# Autodesk Inventor assembly: test
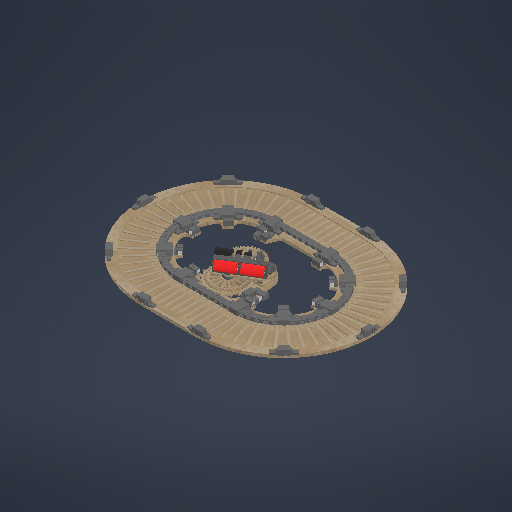
[picture p0: Inventor's stored thumbnail of the model, 512x512]
Saved by Autodesk Inventor 2026.1 (Build 301233020, 233B)
## iProperties
Created: 2025-09-27
Part Number: test
Document SubType Name: Assembly
Designer: hibik
Author: hibik
## Documents named in this file (4)
- C:\Users\hibik\Documents\Robomech\conveyer\All_body.iam
- C:\Users\hibik\Documents\Robomech\conveyer\power_module\Assy_power_module.iam
- C:\Users\hibik\Documents\Robomech\conveyer\liniar_module\linear_module_test.iam
- C:\Users\hibik\Documents\Robomech\conveyer\curve_module\curve_module_test.iam
## Components (11 placed, 3 different names)
1. Assy_power_module:1 [sub-assembly] — フラッシュ:1, 挿入:1, フラッシュ:2, フラッシュ:3
2. linear_module_test:1 [sub-assembly] — 挿入:1, 角度:1, メイト:17, メイト:18, フラッシュ:12
3. curve_module_test:1 [sub-assembly] — メイト:5, メイト:6, フラッシュ:6, メイト:17, メイト:18, フラッシュ:12
4. curve_module_test:2 [sub-assembly] — メイト:5, メイト:6, フラッシュ:6, メイト:9, メイト:10, フラッシュ:8
5. curve_module_test:3 [sub-assembly] — メイト:9, メイト:10, フラッシュ:8
6. curve_module_test:4 [sub-assembly] — メイト:21, メイト:22, フラッシュ:14
7. curve_module_test:5 [sub-assembly] — メイト:19, メイト:20, フラッシュ:13
8. curve_module_test:6 [sub-assembly]
9. curve_module_test:7 [sub-assembly]
10. curve_module_test:8 [sub-assembly]
11. linear_module_test:4 [sub-assembly] — メイト:19, メイト:20, フラッシュ:13, メイト:21, メイト:22, フラッシュ:14
## Relationships (32: Mate 18, Flush 12, Insert 1, Angle 1)
- フラッシュ:1 [Flush]: Assy_power_module:1
- 挿入:1 [Insert] (2.5 mm): Assy_power_module:1 ↔ linear_module_test:1
- 角度:1 [Angle] (0 deg): linear_module_test:1
- フラッシュ:2 [Flush]: Assy_power_module:1
- フラッシュ:3 [Flush]: Assy_power_module:1
- メイト:5 [Mate] (0.5 mm): curve_module_test:1 ↔ curve_module_test:2
- メイト:6 [Mate] (0.5 mm): curve_module_test:1 ↔ curve_module_test:2
- フラッシュ:6 [Flush]: curve_module_test:1 ↔ curve_module_test:2
- [Mate] (0.5 mm): curve_module_test:3 ↔ curve_module_test:4
- [Mate] (0.5 mm): curve_module_test:3 ↔ curve_module_test:4
- [Flush]: curve_module_test:3 ↔ curve_module_test:4
- メイト:9 [Mate] (0.5 mm): curve_module_test:2 ↔ curve_module_test:3
- メイト:10 [Mate] (0.5 mm): curve_module_test:2 ↔ curve_module_test:3
- フラッシュ:8 [Flush]: curve_module_test:2 ↔ curve_module_test:3
- [Mate] (0.5 mm): curve_module_test:5 ↔ curve_module_test:6
- [Mate] (0.5 mm): curve_module_test:5 ↔ curve_module_test:6
- [Flush]: curve_module_test:5 ↔ curve_module_test:6
- [Mate] (0.5 mm): curve_module_test:7 ↔ curve_module_test:8
- [Mate] (0.5 mm): curve_module_test:7 ↔ curve_module_test:8
- [Flush]: curve_module_test:7 ↔ curve_module_test:8
- [Mate] (0.5 mm): curve_module_test:6 ↔ curve_module_test:7
- [Mate] (0.5 mm): curve_module_test:6 ↔ curve_module_test:7
- [Flush]: curve_module_test:6 ↔ curve_module_test:7
- メイト:17 [Mate]: linear_module_test:1 ↔ curve_module_test:1
- メイト:18 [Mate]: linear_module_test:1 ↔ curve_module_test:1
- フラッシュ:12 [Flush]: linear_module_test:1 ↔ curve_module_test:1
- メイト:19 [Mate]: curve_module_test:5 ↔ linear_module_test:4
- メイト:20 [Mate]: curve_module_test:5 ↔ linear_module_test:4
- フラッシュ:13 [Flush]: curve_module_test:5 ↔ linear_module_test:4
- メイト:21 [Mate]: curve_module_test:4 ↔ linear_module_test:4
- メイト:22 [Mate]: curve_module_test:4 ↔ linear_module_test:4
- フラッシュ:14 [Flush]: curve_module_test:4 ↔ linear_module_test:4
## Named parameters: d17_d15 = 0.5 mm, d18_d16 = 0 mm, d19_d14 = 0.5 mm, d23_d15 = 0.5 mm, d24_d16 = 0 mm, d25_d17_d15 = 0.5 mm, d26_d18_d16 = 0 mm, d27_d19_d14 = 0.5 mm, d28_d20 = 0.5 mm, d29_d21 = 0.5 mm, d30_d22 = 0 mm, d31_d14 = 0.5 mm
